# Autodesk Inventor assembly: 花键
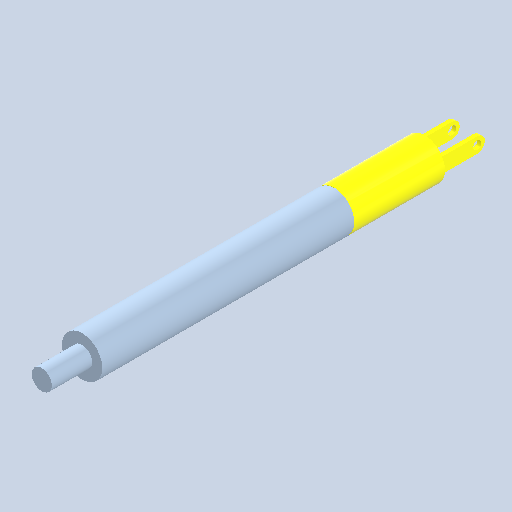
[picture p0: Inventor's stored thumbnail of the model, 512x512]
Saved by Autodesk Inventor 2022 (Build 260153000, 153)
## iProperties
Created: 2023-02-24
Part Number: 花键
Document SubType Name: Assembly
Designer: 李承轩
Author: 李承轩
## Documents named in this file (3)
- D:\Person products\发动机模型\花键.iam
- D:\Person products\发动机模型\传动轴2.ipt
- D:\Person products\发动机模型\节块.ipt
## Components (2 placed, 2 different names)
1. 传动轴2:1 — 插入:1
2. 节块:1 — 插入:1
## Relationships (1: Insert 1)
- 插入:1 [Insert]: 传动轴2:1 ↔ 节块:1
